# Autodesk Inventor assembly: FullCircularAssembly
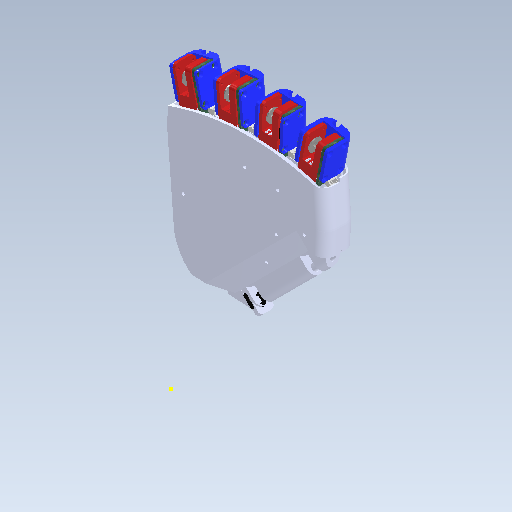
[picture p0: Inventor's stored thumbnail of the model, 512x512]
Saved by Autodesk Inventor 2020 (Build 240168000, 168)
## iProperties
Created: 2020-02-12
Part Number: FullCircularAssembly
Document SubType Name: Assembly
Designer: ttail
Sending System: SolidWorks 2018
Last Author: ttail
Last Saved: 2020-02-15
Author: ttail
## Documents named in this file (13)
- C:\Users\sami_\Documents\V1.6\Workgroups\NotInProject\Palm\FullCircularAssembly.iam
- C:\Users\sami_\Documents\V1.6\Workgroups\NotInProject\UpdatedPartstoSend\Trial Hard surface for circular-Backside.ipt
- C:\Users\sami_\Documents\V1.6\Workgroups\NotInProject\potentiometerbody.ipt
- C:\Users\sami_\Documents\V1.6\Workgroups\NotInProject\Palm\Palm Large Cover.ipt
- C:\Users\sami_\Documents\V1.6\Workgroups\NotInProject\Palm\ActualCircularPalm.ipt
- C:\Users\sami_\Documents\V1.6\Workgroups\NotInProject\Palm\CircularPalmPotCover.ipt
- C:\Users\sami_\Documents\V1.6\Workgroups\NotInProject\Palm\AssemFront2.0.ipt
- C:\Users\sami_\Documents\V1.6\Workgroups\NotInProject\Palm\AssemBack2.0.ipt
- C:\Users\sami_\Documents\V1.6\Workgroups\NotInProject\fingerpanel.ipt
- C:\Users\sami_\Documents\V1.6\Libraries\Content Center Files\en-US\ISO 7089\ISO 7089 - 4 - 140 HV(1).ipt
- C:\Users\sami_\Documents\V1.6\Libraries\Content Center Files\en-US\ISO 1224-1 M\ISO 1224-1 - 17 - 4 x 7 x 2.ipt
- C:\Users\sami_\Documents\V1.6\Libraries\Content Center Files\en-US\ISO 7089\ISO 7089 - 1.6 - 140 HV(1).ipt
- C:\Users\sami_\Documents\V1.6\Workgroups\NotInProject\PotentiometerAssembly.iam
## Components (43 placed, 12 different names)
1. Trial Hard surface for circular-Backside:1 — Mate:54, Mate:55, Mate:78
2. CircularPalmPotCover:1 — Mate:74, Mate:81, Mate:82
3. potentiometerbody:1 — Mate:67, Mate:79, Mate:80
4. ActualCircularPalm:1 — Mate:54, Mate:55, Mate:67, Mate:74, Mate:78, Mate:79, Mate:80, Mate:81, Mate:82, Mate:95, Mate:96, Mate:97, Mate:98, Mate:99, Mate:100, Mate:101, Mate:102, Mate:103, Mate:104, Mate:105
5. Palm Large Cover:1 — Mate:95, Mate:96, Mate:97
6. AssemBack2.0:1 — Mate:102, Mate:103, Mate:104, Mate:105
7. AssemFront2.0:1 — Mate:98, Mate:99, Mate:100, Mate:101
8. fingerpanel:2
9. fingerpanel:4
10. fingerpanel:3
11. fingerpanel:1
12. ISO 7089 4:1
13. ISO 7089 4:2
14. ISO 7089 4:3
15. ISO 7089 4:4
16. ISO 1224-1 (Metric) 17 - 4 x 7 x 2:1
17. ISO 1224-1 (Metric) 17 - 4 x 7 x 2:2
18. ISO 1224-1 (Metric) 17 - 4 x 7 x 2:3
19. ISO 1224-1 (Metric) 17 - 4 x 7 x 2:4
20. ISO 1224-1 (Metric) 17 - 4 x 7 x 2:5
21. ISO 1224-1 (Metric) 17 - 4 x 7 x 2:6
22. ISO 7089 1.6:1
23. ISO 7089 1.6:2
24. ISO 7089 1.6:3
25. ISO 7089 1.6:4
26. ISO 1224-1 (Metric) 17 - 4 x 7 x 2:7
27. ISO 1224-1 (Metric) 17 - 4 x 7 x 2:8
28. ISO 7089 4:5
29. ISO 7089 4:6
30. PotentiometerAssembly:1 [sub-assembly]
31. PotentiometerAssembly:2 [sub-assembly]
32. ISO 7089 1.6:5
33. ISO 7089 1.6:6
34. ISO 7089 1.6:7
35. ISO 7089 1.6:8
36. ISO 7089 1.6:9
37. ISO 7089 1.6:10
38. ISO 7089 1.6:11
39. ISO 7089 1.6:12
40. PotentiometerAssembly:3 [sub-assembly]
41. ISO 7089 4:7
42. ISO 7089 4:8
43. PotentiometerAssembly:4 [sub-assembly]
## Relationships (59: WeldJoint 32, Mate 23, RevoluteJoint 4)
- Mate:54: Trial Hard surface for circular-Backside:1 ↔ ActualCircularPalm:1
- Mate:55: Trial Hard surface for circular-Backside:1 ↔ ActualCircularPalm:1
- Mate:67: potentiometerbody:1 ↔ ActualCircularPalm:1
- Mate:74: CircularPalmPotCover:1 ↔ ActualCircularPalm:1
- Mate:78: Trial Hard surface for circular-Backside:1 ↔ ActualCircularPalm:1
- Mate:79: potentiometerbody:1 ↔ ActualCircularPalm:1
- Mate:80: potentiometerbody:1 ↔ ActualCircularPalm:1
- Mate:81: CircularPalmPotCover:1 ↔ ActualCircularPalm:1
- Mate:82: CircularPalmPotCover:1 ↔ ActualCircularPalm:1
- Mate:95: ActualCircularPalm:1 ↔ Palm Large Cover:1
- Mate:96: ActualCircularPalm:1 ↔ Palm Large Cover:1
- Mate:97: ActualCircularPalm:1 ↔ Palm Large Cover:1
- Mate:98: ActualCircularPalm:1 ↔ AssemFront2.0:1
- Mate:99: ActualCircularPalm:1 ↔ AssemFront2.0:1
- Mate:100: ActualCircularPalm:1 ↔ AssemFront2.0:1
- Mate:101: ActualCircularPalm:1 ↔ AssemFront2.0:1
- Mate:102: ActualCircularPalm:1 ↔ AssemBack2.0:1
- Mate:103: ActualCircularPalm:1 ↔ AssemBack2.0:1
- Mate:104: ActualCircularPalm:1 ↔ AssemBack2.0:1
- Mate:105: ActualCircularPalm:1 ↔ AssemBack2.0:1
- [WeldJoint]: ActualCircularPalm:1 ↔ fingerpanel:3
- [WeldJoint]: ActualCircularPalm:1 ↔ fingerpanel:2
- [WeldJoint]: ActualCircularPalm:1 ↔ fingerpanel:1
- [WeldJoint]: ISO 1224-1 (Metric) 17 - 4 x 7 x 2:8 ↔ ISO 7089 4:5
- [WeldJoint]: PotentiometerAssembly:1 ↔ ISO 7089 1.6:5
- [WeldJoint]: PotentiometerAssembly:1 ↔ ISO 7089 1.6:7
- [WeldJoint]: ISO 7089 4:1 ↔ ISO 1224-1 (Metric) 17 - 4 x 7 x 2:6
- [WeldJoint]: PotentiometerAssembly:2 ↔ ISO 7089 1.6:6
- [WeldJoint]: PotentiometerAssembly:2 ↔ ISO 7089 1.6:8
- [WeldJoint]: PotentiometerAssembly:2 ↔ ISO 7089 1.6:9
- [WeldJoint]: ISO 1224-1 (Metric) 17 - 4 x 7 x 2:7 ↔ ISO 7089 4:6
- [WeldJoint]: ISO 7089 4:4 ↔ ISO 1224-1 (Metric) 17 - 4 x 7 x 2:1
- [WeldJoint]: ISO 7089 4:2 ↔ ISO 1224-1 (Metric) 17 - 4 x 7 x 2:3
- [WeldJoint]: ISO 7089 4:3 ↔ ISO 1224-1 (Metric) 17 - 4 x 7 x 2:5
- [WeldJoint]: ActualCircularPalm:1 ↔ ISO 7089 4:5
- [RevoluteJoint]: ActualCircularPalm:1 ↔ ISO 7089 4:6
- [WeldJoint]: ActualCircularPalm:1 ↔ ISO 7089 4:2
- [RevoluteJoint]: ActualCircularPalm:1 ↔ ISO 7089 4:4
- [WeldJoint]: ActualCircularPalm:1 ↔ ISO 7089 4:1
- [Mate] (0.3 mm): ActualCircularPalm:1 ↔ ISO 7089 1.6:5
- [RevoluteJoint]: ActualCircularPalm:1 ↔ ISO 7089 4:3
- [Mate] (0.3 mm): ActualCircularPalm:1 ↔ ISO 7089 1.6:3
- [WeldJoint] (1.6 mm): ActualCircularPalm:1 ↔ PotentiometerAssembly:1
- [WeldJoint] (1 mm): ActualCircularPalm:1 ↔ PotentiometerAssembly:2
- [WeldJoint]: ISO 7089 1.6:1 ↔ PotentiometerAssembly:3
- [WeldJoint]: ISO 7089 1.6:2 ↔ PotentiometerAssembly:3
- [WeldJoint]: ISO 7089 1.6:3 ↔ PotentiometerAssembly:3
- [WeldJoint]: ISO 7089 1.6:4 ↔ PotentiometerAssembly:3
- [WeldJoint]: PotentiometerAssembly:1 ↔ ISO 7089 1.6:11
- [WeldJoint]: PotentiometerAssembly:1 ↔ ISO 7089 1.6:10
- [WeldJoint]: PotentiometerAssembly:2 ↔ ISO 7089 1.6:12
- [WeldJoint]: ISO 1224-1 (Metric) 17 - 4 x 7 x 2:2 ↔ ISO 7089 4:8
- [WeldJoint]: ISO 1224-1 (Metric) 17 - 4 x 7 x 2:4 ↔ ISO 7089 4:7
- [Mate] (0.3 mm): ActualCircularPalm:1 ↔ ISO 7089 1.6:12
- [WeldJoint]: ActualCircularPalm:1 ↔ ISO 7089 4:8
- [RevoluteJoint]: ActualCircularPalm:1 ↔ ISO 7089 4:7
- [WeldJoint]: fingerpanel:4 ↔ PotentiometerAssembly:3
- [WeldJoint]: ActualCircularPalm:1 ↔ PotentiometerAssembly:3
- [WeldJoint] (1 mm): ActualCircularPalm:1 ↔ PotentiometerAssembly:4
